# Autodesk Inventor assembly: Updated
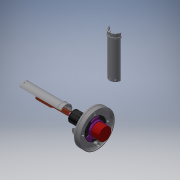
[picture p0: Inventor's stored thumbnail of the model, 180x180]
Saved by Autodesk Inventor 2017 (Build 210142000, 142)
## iProperties
Created: 2017-03-13
Part Number: Updated
Document SubType Name: Assembly
Designer: Joseph
Author: Joseph
## Documents named in this file (16)
- D:\Joseph\Documents\School\College\Clubs\Balloon\2017 Design\Arduino Code\GIT\HELIOS\CAD\Helios.iam
- D:\Joseph\Documents\School\College\Clubs\Balloon\2017 Design\Arduino Code\GIT\HELIOS\CAD\Disc.ipt
- D:\Joseph\Documents\School\College\Clubs\Balloon\2017 Design\Arduino Code\GIT\HELIOS\CAD\LargeO-Ring.ipt
- D:\Joseph\Documents\School\College\Clubs\Balloon\2017 Design\Arduino Code\GIT\HELIOS\CAD\ActuatorCap.ipt
- D:\Joseph\Documents\School\College\Clubs\Balloon\2017 Design\Arduino Code\GIT\HELIOS\CAD\ActuatorRetracted.ipt
- D:\Joseph\Documents\School\College\Clubs\Balloon\2017 Design\Arduino Code\GIT\HELIOS\CAD\Plug.ipt
- D:\Joseph\Documents\School\College\Clubs\Balloon\2017 Design\Arduino Code\GIT\HELIOS\CAD\ValveStem.ipt
- D:\Joseph\Documents\School\College\Clubs\Balloon\2017 Design\Arduino Code\GIT\HELIOS\CAD\ReciprocatingO-Ring.ipt
- D:\Joseph\Documents\School\College\Clubs\Balloon\2017 Design\Arduino Code\GIT\HELIOS\CAD\FillPort.ipt
- D:\Joseph\Documents\School\College\Clubs\Balloon\2017 Design\Arduino Code\GIT\HELIOS\CAD\EyeBolt.ipt
- D:\Joseph\Documents\School\College\Clubs\Balloon\2017 Design\Arduino Code\GIT\HELIOS\CAD\Fan.ipt
- D:\Joseph\Documents\School\College\Clubs\Balloon\2017 Design\Arduino Code\GIT\HELIOS\CAD\FanMount.ipt
- D:\Joseph\Documents\School\College\Clubs\Balloon\2017 Design\Arduino Code\GIT\HELIOS\CAD\FillPlug.ipt
- D:\Joseph\Documents\School\College\Clubs\Balloon\2017 Design\Arduino Code\GIT\HELIOS\CAD\FillPortUpdated.ipt
- D:\Joseph\Documents\School\College\Clubs\Balloon\2017 Design\ExtendedHousingLASide1.ipt
- D:\Joseph\Documents\School\College\Clubs\Balloon\2017 Design\ExtendedHousingLASide2.ipt
## Components (16 placed, 15 different names)
1. Disc:1 — Rigid:1, Rigid:4, Rotational:3, Rotational:4, Rigid:11, Rotational:5
2. LargeO-Ring:1 — Rigid:1
3. ActuatorCap:1 — Rigid:12, Rigid:13
4. ActuatorRetracted:1 — Rigid:12, Mate:1, Mate:2
5. Plug:1 — Rigid:5, Cylindrical:1, Rigid:13
6. ValveStem:1 — Rigid:4, Cylindrical:1, Rigid:9
7. ReciprocatingO-Ring:1 — Rigid:5
8. FillPort:1
9. EyeBolt:1 — Rotational:3
10. EyeBolt:2 — Rotational:4
11. Fan:1 — Rigid:9, Rigid:10
12. FanMount:1 — Rigid:10
13. FillPlug:1 — Rigid:11
14. FillPortUpdated:1 — Rotational:5
15. ExtendedHousingLASide1:1
16. ExtendedHousingLASide2:1 — Mate:1, Mate:2
## Relationships (14: WeldJoint 8, RevoluteJoint 3, Mate 2, CylindricalJoint 1)
- Rigid:1 [WeldJoint] (1.1906 mm): Disc:1 ↔ LargeO-Ring:1
- Rigid:4 [WeldJoint]: Disc:1 ↔ ValveStem:1
- Rigid:5 [WeldJoint]: Plug:1 ↔ ReciprocatingO-Ring:1
- Cylindrical:1: Plug:1 ↔ ValveStem:1
- Rotational:3 [RevoluteJoint] (-5.08 mm): Disc:1 ↔ EyeBolt:1
- Rotational:4 [RevoluteJoint] (-5.08 mm): Disc:1 ↔ EyeBolt:2
- Rigid:9 [WeldJoint]: ValveStem:1 ↔ Fan:1
- Rigid:10 [WeldJoint]: Fan:1 ↔ FanMount:1
- Rigid:11 [WeldJoint]: Disc:1 ↔ FillPlug:1
- Rotational:5 [RevoluteJoint]: Disc:1 ↔ FillPortUpdated:1
- Rigid:12 [WeldJoint]: ActuatorCap:1 ↔ ActuatorRetracted:1
- Rigid:13 [WeldJoint]: ActuatorCap:1 ↔ Plug:1
- Mate:1: ActuatorRetracted:1 ↔ ExtendedHousingLASide2:1
- Mate:2: ActuatorRetracted:1 ↔ ExtendedHousingLASide2:1
